# Autodesk Inventor assembly: beagle_boy
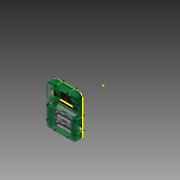
[picture p0: Inventor's stored thumbnail of the model, 180x180]
Saved by Autodesk Inventor 2014 (Build 180170000, 170)
## iProperties
Created: 2013-05-24
Part Number: beagle_boy
Document SubType Name: Assembly
Designer: Administrator
Author: Administrator
## Documents named in this file (21)
- C:\Users\user\Desktop\beagleboy\beagle_boy.iam
- C:\Users\user\Desktop\beagleboy\aaa_holder.ipt
- C:\Users\user\Desktop\beagleboy\Imported Components\Samtec-TSM-123-01-L-DV\Part7.ipt
- C:\Users\user\Desktop\beagleboy\PCB.ipt
- C:\Users\user\Desktop\beagleboy\joystick.ipt
- C:\Users\user\Desktop\beagleboy\button_cap.ipt
- C:\Users\user\Desktop\beagleboy\Imported Components\audio_jack\audio_jack.ipt
- C:\Users\user\Desktop\beagleboy\lcd.iam
- C:\Users\user\Desktop\beagleboy\Imported Components\zif_54\zif_54.ipt
- C:\Users\user\Desktop\beagleboy\beagle_spacer_top.ipt
- C:\Users\user\Desktop\beagleboy\beagle_spacer_bot.ipt
- C:\Users\user\Desktop\beagleboy\beagle_spacer_bot_2.ipt
- C:\Users\user\Desktop\beagleboy\beagle_spacer_bot_3.ipt
- C:\Users\user\Desktop\beagleboy\lid_back.ipt
- C:\Users\user\Desktop\beagleboy\beagle_spacer_bot_4.ipt
- C:\Users\user\Desktop\beagleboy\Imported Components\BEAGLEBONE_BLACK_LS\BEAGLEBONE_BLACK_LS.ipt
- C:\Users\user\Desktop\beagleboy\lcd_spacer.ipt
- C:\Users\user\Desktop\beagleboy\lid_top.ipt
- C:\Users\user\Desktop\beagleboy\Imported Components\standoff_91780A032\standoff_91780A032.ipt
- C:\Users\user\Desktop\beagleboy\Imported Components\screw_black_0.5_91249A058\screw_black_0.5_91249A058.ipt
- C:\Users\user\Desktop\beagleboy\power_switch.ipt
## Components (47 placed, 21 different names)
1. BEAGLEBONE_BLACK_LS:1 — Flush:27, Flush:28, Mate:32, Mate:33, Mate:34
2. aaa_holder:1 — Flush:2, Flush:3, Mate:2, Mate:11, Flush:15
3. aaa_holder:2 — Flush:2, Flush:3, Mate:2
4. Header_1 — Mate:13, Mate:32
5. Header_2 — Mate:12, Mate:33
6. joystick:1 — Mate:18, Angle:7, Mate:39
7. button_cap:1 — Angle:3, Mate:38
8. button_cap:2 — Angle:3, Mate:37
9. audio_jack:1 — Mate:21, Angle:5, Flush:9, Flush:38
10. audio_jack:2 — Mate:22, Angle:4, Flush:10, Flush:37
11. lcd:1 [sub-assembly] — Flush:11, Flush:12
12. zif_54:1 — Mate:24, Angle:6
13. lid_top:1 — Mate:36, Flush:31, Flush:32, Mate:37, Mate:38, Mate:39, Insert:9, Insert:10, Insert:11, Insert:12, Insert:13, Insert:14, Insert:15, Insert:16
14. lcd_spacer:1 — Mate:35, Flush:29, Flush:30, Mate:36
15. PCB:1 — Mate:11, Mate:12, Mate:13, Mate:18, Mate:21, Mate:22, Angle:4, Angle:5, Flush:9, Flush:10, Flush:11, Flush:12, Mate:24, Angle:6, Angle:7, Flush:15, Flush:16, Flush:17, Flush:27, Flush:28, Mate:34, Mate:35, Flush:29, Flush:30, Flush:31, Flush:32, Flush:35, Flush:36, Mate:43, Mate:45, Angle:16, Flush:37, Flush:38
16. beagle_spacer_top:2 — Flush:35, Flush:36, Mate:43, Mate:44
17. beagle_spacer_top:1 — Flush:16, Flush:17, Mate:28, Flush:19, Flush:20, Mate:44
18. beagle_spacer_bot:1 — Mate:28, Flush:19, Flush:20, Flush:21, Flush:22, Mate:29
19. beagle_spacer_bot_2:1 — Flush:21, Flush:22, Mate:29, Mate:30, Flush:23, Flush:24, Angle:8, Angle:9, Angle:10, Angle:11, Angle:12, Angle:13, Angle:14, Angle:15
20. beagle_spacer_bot_3:1 — Mate:30, Flush:23, Flush:24, Mate:31, Flush:25, Flush:26, Insert:1, Insert:2, Insert:3, Insert:4, Insert:5, Insert:6, Insert:7, Insert:8
21. beagle_spacer_bot_4:1 — Mate:31, Flush:25, Flush:26, Mate:42, Flush:33, Flush:34
22. lid_back:1 — Mate:42, Flush:33, Flush:34, Insert:17, Insert:18, Insert:19, Insert:20, Insert:21, Insert:22, Insert:23, Insert:24
23. standoff_91780A032:1 — Insert:2, Angle:9
24. screw_black_0.5_91249A058:1 — Insert:16
25. screw_black_0.5_91249A058:2 — Insert:24
26. screw_black_0.5_91249A058:3 — Insert:9
27. screw_black_0.5_91249A058:4 — Insert:17
28. screw_black_0.5_91249A058:5 — Insert:10
29. screw_black_0.5_91249A058:6 — Insert:18
30. screw_black_0.5_91249A058:7 — Insert:11
31. screw_black_0.5_91249A058:8 — Insert:19
32. screw_black_0.5_91249A058:9 — Insert:12
33. screw_black_0.5_91249A058:10 — Insert:20
34. screw_black_0.5_91249A058:11 — Insert:15
35. screw_black_0.5_91249A058:12 — Insert:21
36. screw_black_0.5_91249A058:13 — Insert:14
37. screw_black_0.5_91249A058:14 — Insert:22
38. screw_black_0.5_91249A058:15 — Insert:13
39. screw_black_0.5_91249A058:16 — Insert:23
40. standoff_91780A032:2 — Insert:8, Angle:15
41. standoff_91780A032:3 — Insert:1, Angle:8
42. standoff_91780A032:4 — Insert:7, Angle:14
43. standoff_91780A032:5 — Insert:6, Angle:13
44. standoff_91780A032:6 — Insert:5, Angle:12
45. standoff_91780A032:7 — Insert:4, Angle:11
46. standoff_91780A032:8 — Insert:3, Angle:10
47. power_switch:1 — Mate:45, Angle:16
## Relationships (94: Flush 29, Mate 27, Insert 24, Angle 14)
- Flush:2: aaa_holder:1 ↔ aaa_holder:2
- Flush:3: aaa_holder:1 ↔ aaa_holder:2
- Mate:2 (0.508 mm): aaa_holder:1 ↔ aaa_holder:2
- Mate:11: aaa_holder:1 ↔ PCB:1
- Mate:12: Header_2 ↔ PCB:1
- Mate:13: Header_1 ↔ PCB:1
- Mate:18: joystick:1 ↔ PCB:1
- Angle:3 (0 deg): button_cap:1 ↔ button_cap:2
- [Mate] (0.9652 mm): button_cap:2 ↔ PCB:1
- [Mate] (0.9652 mm): button_cap:1 ↔ PCB:1
- Mate:21: audio_jack:1 ↔ PCB:1
- Mate:22: audio_jack:2 ↔ PCB:1
- Angle:4 (180 deg): audio_jack:2 ↔ PCB:1
- Angle:5 (180 deg): audio_jack:1 ↔ PCB:1
- Flush:9: audio_jack:1 ↔ PCB:1
- Flush:10: audio_jack:2 ↔ PCB:1
- [Mate] (1.5875 mm): lcd:1 ↔ PCB:1
- Flush:11 (5.969 mm): lcd:1 ↔ PCB:1
- Flush:12 (5.969 mm): lcd:1 ↔ PCB:1
- Mate:24: zif_54:1 ↔ PCB:1
- Angle:6 (180 deg): zif_54:1 ↔ PCB:1
- Angle:7 (180 deg): joystick:1 ↔ PCB:1
- Flush:15 (17.9578 mm): aaa_holder:1 ↔ PCB:1
- Flush:16: PCB:1 ↔ beagle_spacer_top:1
- Flush:17: PCB:1 ↔ beagle_spacer_top:1
- Mate:28: beagle_spacer_top:1 ↔ beagle_spacer_bot:1
- Flush:19: beagle_spacer_top:1 ↔ beagle_spacer_bot:1
- Flush:20: beagle_spacer_top:1 ↔ beagle_spacer_bot:1
- Flush:21: beagle_spacer_bot:1 ↔ beagle_spacer_bot_2:1
- Flush:22: beagle_spacer_bot:1 ↔ beagle_spacer_bot_2:1
- Mate:29: beagle_spacer_bot:1 ↔ beagle_spacer_bot_2:1
- Mate:30: beagle_spacer_bot_2:1 ↔ beagle_spacer_bot_3:1
- Flush:23: beagle_spacer_bot_2:1 ↔ beagle_spacer_bot_3:1
- Flush:24: beagle_spacer_bot_2:1 ↔ beagle_spacer_bot_3:1
- Mate:31: beagle_spacer_bot_3:1 ↔ beagle_spacer_bot_4:1
- Flush:25: beagle_spacer_bot_3:1 ↔ beagle_spacer_bot_4:1
- Flush:26: beagle_spacer_bot_3:1 ↔ beagle_spacer_bot_4:1
- Flush:27: BEAGLEBONE_BLACK_LS:1 ↔ PCB:1
- Flush:28 (12.7 mm): BEAGLEBONE_BLACK_LS:1 ↔ PCB:1
- Mate:32: BEAGLEBONE_BLACK_LS:1 ↔ Header_1
- Mate:33: BEAGLEBONE_BLACK_LS:1 ↔ Header_2
- Mate:34 (0.508 mm): BEAGLEBONE_BLACK_LS:1 ↔ PCB:1
- Mate:35: lcd_spacer:1 ↔ PCB:1
- Flush:29: lcd_spacer:1 ↔ PCB:1
- Flush:30: lcd_spacer:1 ↔ PCB:1
- Mate:36: lid_top:1 ↔ lcd_spacer:1
- Flush:31: lid_top:1 ↔ PCB:1
- Flush:32: lid_top:1 ↔ PCB:1
- Mate:37: button_cap:2 ↔ lid_top:1
- Mate:38: button_cap:1 ↔ lid_top:1
- Mate:39: joystick:1 ↔ lid_top:1
- Insert:1: beagle_spacer_bot_3:1 ↔ standoff_91780A032:3
- Insert:2: beagle_spacer_bot_3:1 ↔ standoff_91780A032:1
- Insert:3: beagle_spacer_bot_3:1 ↔ standoff_91780A032:8
- Insert:4: beagle_spacer_bot_3:1 ↔ standoff_91780A032:7
- Insert:5: beagle_spacer_bot_3:1 ↔ standoff_91780A032:6
- Insert:6: beagle_spacer_bot_3:1 ↔ standoff_91780A032:5
- Insert:7: beagle_spacer_bot_3:1 ↔ standoff_91780A032:4
- Angle:8 (0 deg): beagle_spacer_bot_2:1 ↔ standoff_91780A032:3
- Angle:9 (0 deg): beagle_spacer_bot_2:1 ↔ standoff_91780A032:1
- Angle:10 (0 deg): beagle_spacer_bot_2:1 ↔ standoff_91780A032:8
- Angle:11 (0 deg): beagle_spacer_bot_2:1 ↔ standoff_91780A032:7
- Angle:12 (0 deg): beagle_spacer_bot_2:1 ↔ standoff_91780A032:6
- Angle:13 (0 deg): beagle_spacer_bot_2:1 ↔ standoff_91780A032:5
- Angle:14 (0 deg): beagle_spacer_bot_2:1 ↔ standoff_91780A032:4
- Insert:8: beagle_spacer_bot_3:1 ↔ standoff_91780A032:2
- Angle:15 (0 deg): beagle_spacer_bot_2:1 ↔ standoff_91780A032:2
- Insert:9: lid_top:1 ↔ screw_black_0.5_91249A058:3
- Insert:10: lid_top:1 ↔ screw_black_0.5_91249A058:5
- Insert:11: lid_top:1 ↔ screw_black_0.5_91249A058:7
- Insert:12: lid_top:1 ↔ screw_black_0.5_91249A058:9
- Insert:13: lid_top:1 ↔ screw_black_0.5_91249A058:15
- Insert:14: lid_top:1 ↔ screw_black_0.5_91249A058:13
- Insert:15: lid_top:1 ↔ screw_black_0.5_91249A058:11
- Insert:16: lid_top:1 ↔ screw_black_0.5_91249A058:1
- Mate:42: beagle_spacer_bot_4:1 ↔ lid_back:1
- Flush:33: beagle_spacer_bot_4:1 ↔ lid_back:1
- Flush:34: beagle_spacer_bot_4:1 ↔ lid_back:1
- Insert:17: lid_back:1 ↔ screw_black_0.5_91249A058:4
- Insert:18: lid_back:1 ↔ screw_black_0.5_91249A058:6
- Insert:19: lid_back:1 ↔ screw_black_0.5_91249A058:8
- Insert:20: lid_back:1 ↔ screw_black_0.5_91249A058:10
- Insert:21: lid_back:1 ↔ screw_black_0.5_91249A058:12
- Insert:22: lid_back:1 ↔ screw_black_0.5_91249A058:14
- Insert:23: lid_back:1 ↔ screw_black_0.5_91249A058:16
- Insert:24: lid_back:1 ↔ screw_black_0.5_91249A058:2
- Flush:35: PCB:1 ↔ beagle_spacer_top:2
- Flush:36: PCB:1 ↔ beagle_spacer_top:2
- Mate:43: PCB:1 ↔ beagle_spacer_top:2
- Mate:44: beagle_spacer_top:2 ↔ beagle_spacer_top:1
- Mate:45: PCB:1 ↔ power_switch:1
- Angle:16 (0 deg): PCB:1 ↔ power_switch:1
- Flush:37: audio_jack:2 ↔ PCB:1
- Flush:38: audio_jack:1 ↔ PCB:1
